# Autodesk Inventor assembly: LegMiddle
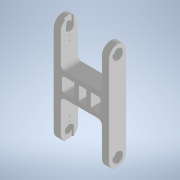
[picture p0: Inventor's stored thumbnail of the model, 180x180]
Saved by Autodesk Inventor 2020.3 (Build 243373000, 373)
## iProperties
Created: 2022-04-03
Part Number: LegMiddle
Document SubType Name: Assembly
Designer: sanyi
Author: sanyi
## Documents named in this file (2)
- C:\Users\sanyi\Documents\Inventor\Quadropod\Quadropod MDL\SimulationModell_Assembly\LegMiddle.iam
- C:\Users\sanyi\Documents\Inventor\Quadropod\Quadropod MDL\SimulationModell_Assembly\LegMiddle.ipt
## Components (1 placed, 1 different names)
1. LegMiddle:1 — Mate:2, Mate:3, Flush:1
## Relationships (3: Mate 2, Flush 1)
- Mate:2: LegMiddle:1
- Mate:3: LegMiddle:1
- Flush:1: LegMiddle:1
